# Autodesk Inventor assembly: LED_Strip_mit_Halter
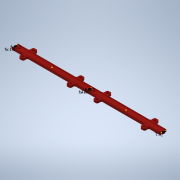
[picture p0: Inventor's stored thumbnail of the model, 180x180]
Saved by Autodesk Inventor 2021.2 (Build 252289000, 289)
## iProperties
Company: Schneeberger Lineartechnik AG
RuleStatus: InUse
Created: 2021-09-27
Part Number: LED_Strip_mit_Halter
User Status: Schnelländerung
Document SubType Name: Assembly
Designer: SRORF
Mass: 38.4195 g
Surface Area: 263.127 cm^2
Volume: 33.9835 cm^3
Density: 1.13053 g/cm^3
Status: Produktion Freigegeben
ROT_Density: 0.0
PDB_Ident_Ver: =<PDB_Ident> <PDB_Version>
ROT_Weight: 0.038 kg
ROT_Weight_Num: 0.03841945576225316
Author: SRORF
## Documents named in this file (3)
- D:\Dropbox\Dropbox\Uhr\3D_Daten\CAD\LED_Strip_mit_Halter.iam
- D:\Dropbox\Dropbox\Uhr\3D_Daten\CAD\LED_Strip_Halter.ipt
- D:\Dropbox\Dropbox\Uhr\3D_Daten\CAD\LED_Strip.iam
## Components (3 placed, 2 different names)
1. --:30 [sub-assembly] — Passend:1, Passend:3, Fluchtend:1
2. --:28 — Passend:1, Passend:3, Passend:4, Passend:5, Passend:6
3. LED_Strip_Halter:2
## Component patterns: (2 elements, first: --:28)
## Relationships (6: Mate 5, Flush 1)
- Passend:1 [Mate]: --:30 ↔ --:28
- Passend:3 [Mate]: --:30 ↔ --:28
- Passend:4 [Mate]: --:28
- Passend:5 [Mate]: --:28
- Passend:6 [Mate]: --:28
- Fluchtend:1 [Flush]: --:30
